# Autodesk Inventor assembly: BC-100003_Base maior
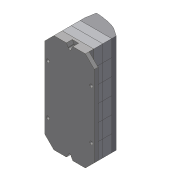
[picture p0: Inventor's stored thumbnail of the model, 180x180]
Saved by Autodesk Inventor 2016 (Build 200138000, 138)
## iProperties
Created: 2015-09-23
Part Number: BC-100003_Base maior
Document SubType Name: Assembly
Designer: Reinaldo.Basílio
Mass: 35341.7 g
Surface Area: 4837.15 cm^2
Volume: 4562.02 cm^3
Density: 7.74696 g/cm^3
Author: Reinaldo.Basílio
## Documents named in this file (4)
- D:\ARQ\Basilio\LNLS-2\Anel\Dipolos\Dipolo 2T\Dipolo 3T e 1T\Prototipo 1\Desenhos\BC-100003_Base maior.iam
- D:\ARQ\Basilio\LNLS-2\Anel\Dipolos\Dipolo 2T\Dipolo 3T e 1T\Prototipo 1\Desenhos\BC-100002.iam
- D:\ARQ\Basilio\LNLS-2\Anel\Dipolos\Dipolo 2T\Dipolo 3T e 1T\Prototipo 1\Desenhos\BC-10005.ipt
- D:\ARQ\Basilio\LNLS-2\Anel\Dipolos\Dipolo 2T\Dipolo 3T e 1T\Prototipo 1\Desenhos\BC-10008_B.ipt
## Components (3 placed, 3 different names)
1. BC-10005:1 — Flush:10, Mate:4, Mate:5, Flush:12, Mate:6, Flush:13
2. BC-100002:1 [sub-assembly] — Mate:2, Flush:7, Flush:11, Mate:6
3. BC-10008_B:1 — Mate:2, Flush:7, Flush:11, Flush:12, Flush:13
## Relationships (9: Flush 5, Mate 4)
- Mate:2: BC-100002:1 ↔ BC-10008_B:1
- Flush:7: BC-100002:1 ↔ BC-10008_B:1
- Flush:10: BC-10005:1
- Mate:4: BC-10005:1
- Mate:5: BC-10005:1
- Flush:11: BC-100002:1 ↔ BC-10008_B:1
- Flush:12: BC-10005:1 ↔ BC-10008_B:1
- Mate:6: BC-10005:1 ↔ BC-100002:1
- Flush:13: BC-10005:1 ↔ BC-10008_B:1
